# Autodesk Inventor assembly: odom_pod
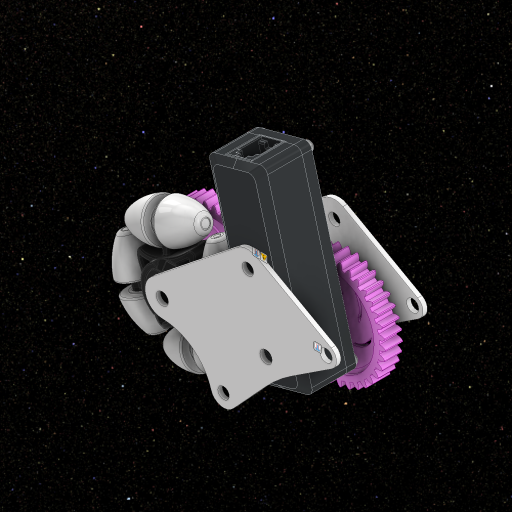
[picture p0: Inventor's stored thumbnail of the model, 512x512]
Saved by Autodesk Inventor 2024 (Build 280153000, 153)
## iProperties
Created: 2024-02-24
Part Number: odom_pod
Document SubType Name: Assembly
Designer: Averey Ku
Author: Averey Ku
## Documents named in this file (5)
- D:\vex_robotics\hardware\cad\vroomba_v0.1\odom_pod.iam
- C:\Users\Averey Ku\Downloads\2” Omni-Directional Wheel (276-9044)\2” Omni-Directional Wheel (276-9044).ipt
- D:\vex_robotics\hardware\cad\vroomba_v0.1\odom_pod.ipt
- D:\vex_robotics\hardware\cad\VEX-CAD-Inventor-1.41\Electronics\Sensors\V5 Rotation Sensor.ipt
- D:\vex_robotics\hardware\cad\VEX-CAD-Inventor-1.41\Motion\Gears\LS 36T Gear.ipt
## Components (6 placed, 4 different names)
1. 2” Omni-Directional Wheel (276-9044):1 — Insert:2, Insert:5
2. odom_pod:1 — Insert:1, Insert:2, Mate:2, Mate:3, Insert:7
3. V5 Rotation Sensor:1 — Insert:1, Mate:2, Mate:3, Insert:4
4. LS 36T Gear:1 — Insert:4
5. LS 36T Gear:2 — Insert:5, Insert:6
6. odom_pod:2 — Insert:6, Insert:7
## Relationships (8: Insert 6, Mate 2)
- Insert:1: odom_pod:1 ↔ V5 Rotation Sensor:1
- Insert:2: 2” Omni-Directional Wheel (276-9044):1 ↔ odom_pod:1
- Mate:2: odom_pod:1 ↔ V5 Rotation Sensor:1
- Mate:3: odom_pod:1 ↔ V5 Rotation Sensor:1
- Insert:4: V5 Rotation Sensor:1 ↔ LS 36T Gear:1
- Insert:5: 2” Omni-Directional Wheel (276-9044):1 ↔ LS 36T Gear:2
- Insert:6 (6.35 mm): LS 36T Gear:2 ↔ odom_pod:2
- Insert:7 (30.1625 mm): odom_pod:1 ↔ odom_pod:2
